# Autodesk Inventor assembly: ALL
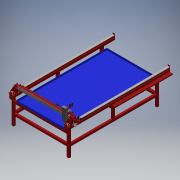
[picture p0: Inventor's stored thumbnail of the model, 180x180]
Saved by Autodesk Inventor 2018.2 (Build 222227000, 227)
## iProperties
Created: 2017-12-19
Part Number: ALL
Document SubType Name: Assembly
Designer: torba
Author: torba
## Documents named in this file (7)
- C:\Users\torba\OneDrive\Documents\Inventor\Plasma 5x10\ALL.iam
- C:\Users\torba\OneDrive\Documents\Inventor\Plasma 5x10\Lower Frame.iam
- C:\Users\torba\OneDrive\Documents\Inventor\Plasma 5x10\Gantry.iam
- C:\Users\torba\OneDrive\Documents\Inventor\Plasma 5x10\z.iam
- C:\Users\torba\OneDrive\Documents\Inventor\Plasma 5x10\Water Table.iam
- C:\Users\torba\OneDrive\Documents\Inventor\Plasma 5x10\C4 Channel\C4 Channel-81.ipt
- C:\Users\torba\OneDrive\Documents\Inventor\Plasma 5x10\C4 Channel.ipt
## Components (5 placed, 5 different names)
1. Lower Frame:1 [sub-assembly] — Angle:1, Mate:1, Mate:2, Flush:1, Mate:3, Tangent:1, Mate:4, Flush:3, Mate:5, Mate:6
2. Gantry:1 [sub-assembly] — Angle:1, Mate:1, Tangent:1, Tangent:2, Tangent:3, Flush:2, Mate:6, Mate:7
3. z:1 [sub-assembly] — Tangent:2, Tangent:3, Flush:2, Mate:7
4. Water Table:1 [sub-assembly] — Mate:2, Flush:1, Mate:3
5. C4 Channel-81:1 — Mate:4, Flush:3, Mate:5
## Relationships (14: Mate 7, Flush 3, Tangent 3, Angle 1)
- Angle:1 (0 deg): Lower Frame:1 ↔ Gantry:1
- Mate:1 (6.35 mm): Lower Frame:1 ↔ Gantry:1
- Mate:2: Lower Frame:1 ↔ Water Table:1
- Flush:1: Lower Frame:1 ↔ Water Table:1
- Mate:3 (101.6 mm): Lower Frame:1 ↔ Water Table:1
- Tangent:1: Lower Frame:1 ↔ Gantry:1
- Tangent:2: Gantry:1 ↔ z:1
- Tangent:3: Gantry:1 ↔ z:1
- Flush:2 (0.3556 mm): Gantry:1 ↔ z:1
- Mate:4: Lower Frame:1 ↔ C4 Channel-81:1
- Flush:3 (76.2 mm): Lower Frame:1 ↔ C4 Channel-81:1
- Mate:5: Lower Frame:1 ↔ C4 Channel-81:1
- Mate:6: Lower Frame:1 ↔ Gantry:1
- Mate:7: Gantry:1 ↔ z:1
